# Autodesk Inventor assembly: Assembly2
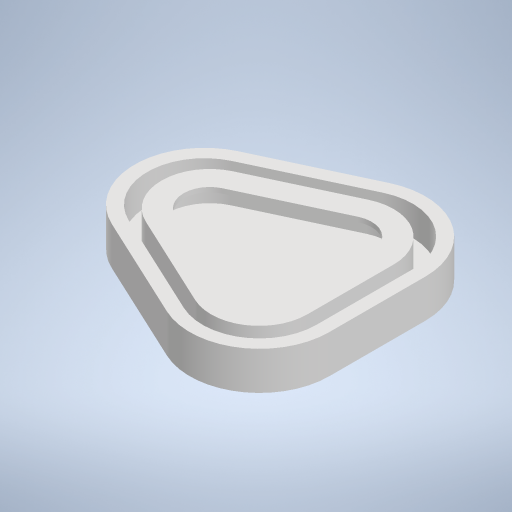
[picture p0: Inventor's stored thumbnail of the model, 512x512]
Saved by Autodesk Inventor 2024.3 (Build 283343000, 343)
## iProperties
Created: 2025-06-26
Part Number: Assembly2
Document SubType Name: Assembly
Designer: 1
Author: 1
## Documents named in this file (3)
- F:\UMN Researches\CUHK Research\SKIN\Assembly2.iam
- F:\UMN Researches\CUHK Research\SKIN\Tri_Box.ipt
- F:\UMN Researches\CUHK Research\SKIN\Magne_Cover.ipt
## Components (2 placed, 2 different names)
1. Tri_Box:1 — Mate:1, Mate:2, Mate:3
2. Magne_Cover:1 — Mate:1, Mate:2, Mate:3
## Relationships (3: Mate 3)
- Mate:1: Tri_Box:1 ↔ Magne_Cover:1
- Mate:2 (3 mm): Tri_Box:1 ↔ Magne_Cover:1
- Mate:3 (3 mm): Tri_Box:1 ↔ Magne_Cover:1
